# Autodesk Inventor assembly: gripper_finger
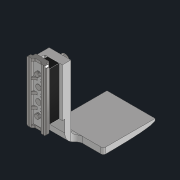
[picture p0: Inventor's stored thumbnail of the model, 180x180]
Saved by Autodesk Inventor 2022 (Build 260153000, 153)
## iProperties
Created: 2021-10-20
Part Number: gripper_finger
Document SubType Name: Assembly
Designer: Yuta Kage
Author: Yuta Kage
## Documents named in this file (5)
- C:\Users\yuta0\Documents\GitHub\catchrobo_hardware\mesh\scara\gripper_finger.iam
- C:\Users\yuta0\Documents\GitHub\catchrobo_hardware\assy-scara\mr-20cs_1.iam
- C:\Users\yuta0\Documents\GitHub\catchrobo_hardware\assy-scara\base37.ipt
- C:\Users\yuta0\Documents\GitHub\catchrobo_hardware\assy-scara\base49.ipt
- C:\Users\yuta0\Documents\GitHub\catchrobo_hardware\assy-scara\CB4-20.ipt
## Components (5 placed, 4 different names)
1. base37:1 — メイト:2, メイト:3, メイト:4, メイト:11
2. base49:1 — メイト:1, メイト:2, メイト:3, メイト:4, メイト:5, メイト:6, メイト:7, メイト:8, メイト:12, フラッシュ:1
3. CB4-20:1 — メイト:5, メイト:8, メイト:10
4. CB4-20:2 — メイト:6, メイト:7, メイト:9
5. mr-20cs_1:1 [sub-assembly] — メイト:9, メイト:10, メイト:11
## Relationships (13: Mate 12, Flush 1)
- メイト:1 [Mate] (-20 mm): base49:1
- メイト:2 [Mate]: base37:1 ↔ base49:1
- メイト:3 [Mate]: base37:1 ↔ base49:1
- メイト:4 [Mate]: base37:1 ↔ base49:1
- メイト:5 [Mate]: base49:1 ↔ CB4-20:1
- メイト:6 [Mate]: base49:1 ↔ CB4-20:2
- メイト:7 [Mate]: base49:1 ↔ CB4-20:2
- メイト:8 [Mate]: base49:1 ↔ CB4-20:1
- メイト:9 [Mate]: CB4-20:2 ↔ mr-20cs_1:1
- メイト:10 [Mate]: CB4-20:1 ↔ mr-20cs_1:1
- メイト:11 [Mate]: base37:1 ↔ mr-20cs_1:1
- メイト:12 [Mate]: base49:1
- フラッシュ:1 [Flush]: base49:1
